# Autodesk Inventor assembly: Assembly_Trial_3
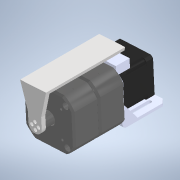
[picture p0: Inventor's stored thumbnail of the model, 180x180]
Saved by Autodesk Inventor 2022 (Build 260153000, 153)
## iProperties
Created: 2022-01-15
Part Number: Assembly_Trial_3
Document SubType Name: Assembly
Designer: Mlees
Author: Mlees
## Documents named in this file (13)
- C:\Users\Mlees\Desktop\504_Engineering\Stepper-Servo_Based_Robotic_Arm\Assembly_Trial_3.iam
- C:\Users\Mlees\Desktop\504_Engineering\Stepper-Servo_Based_Robotic_Arm\Downloaded Parts\nema17-speed-reducer-1.snapshot.9\24_Teeth_Sun_Gear.step.ipt
- C:\Users\Mlees\Desktop\504_Engineering\Stepper-Servo_Based_Robotic_Arm\Downloaded Parts\nema17-speed-reducer-1.snapshot.9\36_Teeth_Planet_Gear.step.ipt
- C:\Users\Mlees\Desktop\504_Engineering\Stepper-Servo_Based_Robotic_Arm\Downloaded Parts\nema17-speed-reducer-1.snapshot.9\96_Teeth_Gear.step.ipt
- C:\Users\Mlees\Desktop\504_Engineering\Stepper-Servo_Based_Robotic_Arm\Downloaded Parts\nema17-speed-reducer-1.snapshot.9\Gear_Cover.ipt
- C:\Users\Mlees\Desktop\504_Engineering\Stepper-Servo_Based_Robotic_Arm\Downloaded Parts\nema17-speed-reducer-1.snapshot.9\Plamet_Carrier.ipt
- C:\Users\Mlees\Desktop\504_Engineering\Stepper-Servo_Based_Robotic_Arm\Downloaded Parts\90751A113_18-8 Stainless Steel Socket Head Screws.ipt
- C:\Users\Mlees\Desktop\504_Engineering\Stepper-Servo_Based_Robotic_Arm\Downloaded Parts\nema-17-motor-mount-1.snapshot.1\NEMA_17_Bracket.ipt
- C:\Users\Mlees\Desktop\504_Engineering\Stepper-Servo_Based_Robotic_Arm\Downloaded Parts\nema17-speed-reducer-1.snapshot.9\Thread Insert M3 x 6mm v2.step.iam
- C:\Users\Mlees\Desktop\504_Engineering\Stepper-Servo_Based_Robotic_Arm\Downloaded Parts\Harmonic_Drive\Nema 17.ipt
- C:\Users\Mlees\Desktop\504_Engineering\Stepper-Servo_Based_Robotic_Arm\Downloaded Parts\nema17-speed-reducer-1.snapshot.9\Gear_Cover_modified.ipt
- C:\Users\Mlees\Desktop\504_Engineering\Stepper-Servo_Based_Robotic_Arm\Downloaded Parts\nema17-speed-reducer-1.snapshot.9\Plamet_Carrier_modified.ipt
- C:\Users\Mlees\Desktop\504_Engineering\Stepper-Servo_Based_Robotic_Arm\Created Parts\OutPut_Shaft_From_Gearbox.ipt
## Components (40 placed, 12 different names)
1. 24_Teeth_Sun_Gear.step:1 — Rotational:6, Rotational:11
2. 36_Teeth_Planet_Gear.step:1 — Rotational:3
3. 96_Teeth_Gear.step:1 — Rigid:2, Rigid:3, Rigid:4, Rigid:5, Rotational:7, Rotational:8, Rotational:9, Rotational:10, Rigid:7
4. Gear_Cover:1 — Rigid:7, Rigid:8, Rigid:9, Rigid:10, Rigid:11, Rigid:13
5. Plamet_Carrier:1 — Rotational:3, Rotational:4, Rotational:5, Rotational:6, Rotational:23, Rotational:24
6. 90751A113_18-8 Stainless Steel Socket Head Screws:1 — Rigid:3
7. 90751A113_18-8 Stainless Steel Socket Head Screws:2 — Rigid:4
8. 90751A113_18-8 Stainless Steel Socket Head Screws:3 — Rigid:5
9. NEMA_17_Bracket:1 — Rigid:2, Rigid:12
10. 36_Teeth_Planet_Gear.step:2 — Rotational:4
11. 36_Teeth_Planet_Gear.step:4 — Rotational:5
12. Thread Insert M3 x 6mm v2.step:1 [sub-assembly] — Rotational:7
13. Thread Insert M3 x 6mm v2.step:2 [sub-assembly] — Rotational:8
14. Thread Insert M3 x 6mm v2.step:3 [sub-assembly] — Rotational:9
15. Thread Insert M3 x 6mm v2.step:4 [sub-assembly] — Rotational:10
16. 90751A113_18-8 Stainless Steel Socket Head Screws:4 — Rigid:8
17. 90751A113_18-8 Stainless Steel Socket Head Screws:5 — Rigid:9
18. 90751A113_18-8 Stainless Steel Socket Head Screws:6 — Rigid:10
19. 90751A113_18-8 Stainless Steel Socket Head Screws:7 — Rigid:11
20. Nema 17:1 — Rigid:12, Rotational:11
21. 96_Teeth_Gear.step:2 — Rigid:13, Rotational:12, Rotational:13, Rotational:14, Rotational:15, Rotational:16, Rotational:17, Rotational:18, Rotational:19, Rigid:14
22. 90751A113_18-8 Stainless Steel Socket Head Screws:8 — Rotational:12
23. 90751A113_18-8 Stainless Steel Socket Head Screws:9 — Rotational:15
24. 90751A113_18-8 Stainless Steel Socket Head Screws:10 — Rotational:14
25. 90751A113_18-8 Stainless Steel Socket Head Screws:11 — Rotational:13
26. Thread Insert M3 x 6mm v2.step:5 [sub-assembly] — Rotational:16
27. Thread Insert M3 x 6mm v2.step:6 [sub-assembly] — Rotational:18
28. Thread Insert M3 x 6mm v2.step:7 [sub-assembly] — Rotational:19
29. Thread Insert M3 x 6mm v2.step:8 [sub-assembly] — Rotational:17
30. 24_Teeth_Sun_Gear.step:2 — Rotational:23
31. 36_Teeth_Planet_Gear.step:5
32. 36_Teeth_Planet_Gear.step:6
33. 36_Teeth_Planet_Gear.step:7
34. 90751A113_18-8 Stainless Steel Socket Head Screws:12
35. 90751A113_18-8 Stainless Steel Socket Head Screws:13
36. 90751A113_18-8 Stainless Steel Socket Head Screws:14
37. 90751A113_18-8 Stainless Steel Socket Head Screws:15
38. Gear_Cover_modified:1 — Rigid:14
39. Plamet_Carrier_modified:1 — Rotational:24, Rigid:15
40. OutPut_Shaft_From_Gearbox:1 — Rigid:15
## Relationships (32: RevoluteJoint 19, WeldJoint 13)
- Rigid:2 [WeldJoint]: 96_Teeth_Gear.step:1 ↔ NEMA_17_Bracket:1
- Rigid:3 [WeldJoint]: 96_Teeth_Gear.step:1 ↔ 90751A113_18-8 Stainless Steel Socket Head Screws:1
- Rigid:4 [WeldJoint]: 96_Teeth_Gear.step:1 ↔ 90751A113_18-8 Stainless Steel Socket Head Screws:2
- Rigid:5 [WeldJoint]: 96_Teeth_Gear.step:1 ↔ 90751A113_18-8 Stainless Steel Socket Head Screws:3
- Rotational:3 [RevoluteJoint]: 36_Teeth_Planet_Gear.step:1 ↔ Plamet_Carrier:1
- Rotational:4 [RevoluteJoint]: Plamet_Carrier:1 ↔ 36_Teeth_Planet_Gear.step:2
- Rotational:5 [RevoluteJoint]: Plamet_Carrier:1 ↔ 36_Teeth_Planet_Gear.step:4
- Rotational:6 [RevoluteJoint]: 24_Teeth_Sun_Gear.step:1 ↔ Plamet_Carrier:1
- Rotational:7 [RevoluteJoint]: 96_Teeth_Gear.step:1 ↔ Thread Insert M3 x 6mm v2.step:1
- Rotational:8 [RevoluteJoint]: 96_Teeth_Gear.step:1 ↔ Thread Insert M3 x 6mm v2.step:2
- Rotational:9 [RevoluteJoint]: 96_Teeth_Gear.step:1 ↔ Thread Insert M3 x 6mm v2.step:3
- Rotational:10 [RevoluteJoint]: 96_Teeth_Gear.step:1 ↔ Thread Insert M3 x 6mm v2.step:4
- Rigid:7 [WeldJoint]: 96_Teeth_Gear.step:1 ↔ Gear_Cover:1
- Rigid:8 [WeldJoint]: Gear_Cover:1 ↔ 90751A113_18-8 Stainless Steel Socket Head Screws:4
- Rigid:9 [WeldJoint]: Gear_Cover:1 ↔ 90751A113_18-8 Stainless Steel Socket Head Screws:5
- Rigid:10 [WeldJoint]: Gear_Cover:1 ↔ 90751A113_18-8 Stainless Steel Socket Head Screws:6
- Rigid:11 [WeldJoint]: Gear_Cover:1 ↔ 90751A113_18-8 Stainless Steel Socket Head Screws:7
- Rigid:12 [WeldJoint]: NEMA_17_Bracket:1 ↔ Nema 17:1
- Rotational:11 [RevoluteJoint]: 24_Teeth_Sun_Gear.step:1 ↔ Nema 17:1
- Rigid:13 [WeldJoint]: Gear_Cover:1 ↔ 96_Teeth_Gear.step:2
- Rotational:12 [RevoluteJoint]: 96_Teeth_Gear.step:2 ↔ 90751A113_18-8 Stainless Steel Socket Head Screws:8
- Rotational:13 [RevoluteJoint]: 96_Teeth_Gear.step:2 ↔ 90751A113_18-8 Stainless Steel Socket Head Screws:11
- Rotational:14 [RevoluteJoint]: 96_Teeth_Gear.step:2 ↔ 90751A113_18-8 Stainless Steel Socket Head Screws:10
- Rotational:15 [RevoluteJoint]: 96_Teeth_Gear.step:2 ↔ 90751A113_18-8 Stainless Steel Socket Head Screws:9
- Rotational:16 [RevoluteJoint]: 96_Teeth_Gear.step:2 ↔ Thread Insert M3 x 6mm v2.step:5
- Rotational:17 [RevoluteJoint]: 96_Teeth_Gear.step:2 ↔ Thread Insert M3 x 6mm v2.step:8
- Rotational:18 [RevoluteJoint]: 96_Teeth_Gear.step:2 ↔ Thread Insert M3 x 6mm v2.step:6
- Rotational:19 [RevoluteJoint]: 96_Teeth_Gear.step:2 ↔ Thread Insert M3 x 6mm v2.step:7
- Rotational:23 [RevoluteJoint]: Plamet_Carrier:1 ↔ 24_Teeth_Sun_Gear.step:2
- Rotational:24 [RevoluteJoint]: Plamet_Carrier:1 ↔ Plamet_Carrier_modified:1
- Rigid:14 [WeldJoint]: 96_Teeth_Gear.step:2 ↔ Gear_Cover_modified:1
- Rigid:15 [WeldJoint]: Plamet_Carrier_modified:1 ↔ OutPut_Shaft_From_Gearbox:1
